# Autodesk Inventor assembly: am_6375
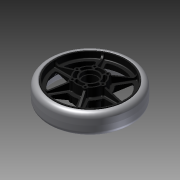
[picture p0: Inventor's stored thumbnail of the model, 180x180]
Saved by Autodesk Inventor 2011 (Build 150239000, 239)
## iProperties
Category: Drive Train
Company: Autodesk Inc.
Created: 2008-12-09
Part Number: am_6375
Document SubType Name: Assembly
Designer: Autodesk Inc.
Catalog Web Link: http://andymark.biz/index.html
Vendor: Andy Mark Inc.
Author: Autodesk Inc.
## Documents named in this file (3)
- R:\2012\Inventor\vkop\All-Drive-Train\Wheel_AndyMark_am_6375.iam
- R:\2012\Inventor\vkop\All-Drive-Train\6 wheel IIA.ipt
- R:\2012\Inventor\vkop\All-Drive-Train\First 09 Wheel_6+375 tread Simple.ipt
## Components (2 placed, 2 different names)
1. 6 wheel IIA:1 — Insert:1
2. First 09 Wheel_6+375 tread Simple:1 — Insert:1
## Relationships (1: Insert 1)
- Insert:1: 6 wheel IIA:1 ↔ First 09 Wheel_6+375 tread Simple:1
